# Autodesk Inventor assembly: 4 Pin Male
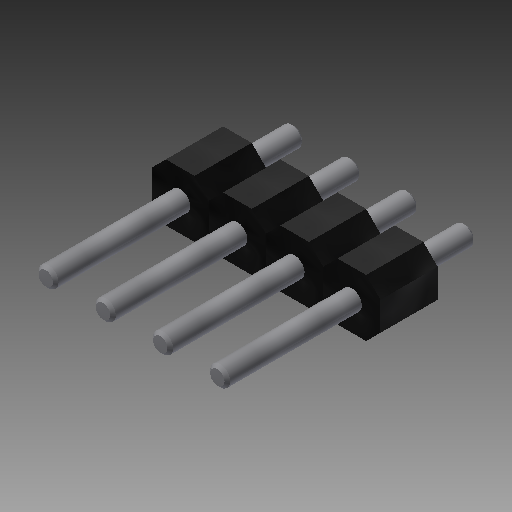
[picture p0: Inventor's stored thumbnail of the model, 512x512]
Saved by Autodesk Inventor 2017 (Build 210142000, 142)
## iProperties
Created: 2016-08-16
Part Number: 4 Pin Male
Document SubType Name: Assembly
Designer: ge937963
Author: ge937963
## Documents named in this file (2)
- Z:\allusers\Diagnostics\Inventor Files\3dPrintedPCR\4 Pin Male.iam
- Z:\allusers\Diagnostics\Inventor Files\3dPrintedPCR\Pin.ipt
## Components (4 placed, 1 different names)
1. Pin:1 — Flush:1, Flush:4, Mate:1
2. Pin:2 — Flush:1, Flush:2, Flush:4, Flush:5, Mate:1, Mate:2
3. Pin:3 — Flush:2, Flush:3, Flush:5, Flush:6, Mate:2, Mate:3
4. Pin:4 — Flush:3, Flush:6, Mate:3
## Relationships (9: Flush 6, Mate 3)
- Flush:1: Pin:1 ↔ Pin:2
- Flush:2: Pin:2 ↔ Pin:3
- Flush:3: Pin:3 ↔ Pin:4
- Flush:4: Pin:1 ↔ Pin:2
- Flush:5: Pin:2 ↔ Pin:3
- Flush:6: Pin:3 ↔ Pin:4
- Mate:1: Pin:1 ↔ Pin:2
- Mate:2: Pin:2 ↔ Pin:3
- Mate:3: Pin:3 ↔ Pin:4
